# Autodesk Inventor assembly: ArmWithBase
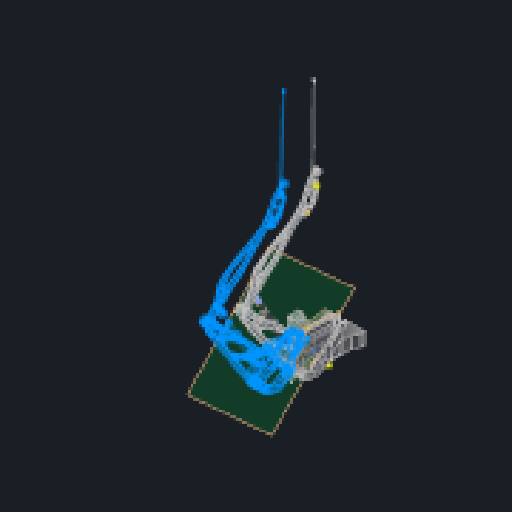
[picture p0: Inventor's stored thumbnail of the model, 512x512]
Saved by Autodesk Inventor 2025.2 (Build 292293000, 293)
## iProperties
Created: 2025-01-19
Part Number: ArmWithBase
Document SubType Name: Assembly
Designer: valer
Author: valer
## Documents named in this file (4)
- C:\Users\valer\Desktop\str1ker\cad\ArmFrontRight.iam
- C:\Users\valer\Desktop\str1ker\cad\ArmBase.iam
- C:\Users\valer\Desktop\str1ker\cad\Arm.iam
- C:\Users\valer\Desktop\str1ker\cad\ArmScapula.ipt
## Components (4 placed, 3 different names)
1. Base:1 [sub-assembly] — Mate:5, Mate:6, Mate:7, Mate:9, Mate:13, Mate:14, Mate:15
2. Arm:1 [sub-assembly] — Mate:5, Mate:6, Mate:8
3. ArmScapula:1 — Mate:9
4. ArmScapula:2 — Mate:13, Mate:14, Mate:15
## Relationships (8: Mate 8)
- Mate:5: Base:1 ↔ Arm:1
- Mate:6: Base:1 ↔ Arm:1
- Mate:7: Base:1
- Mate:8: Arm:1
- Mate:9: Base:1 ↔ ArmScapula:1
- Mate:13: Base:1 ↔ ArmScapula:2
- Mate:14: Base:1 ↔ ArmScapula:2
- Mate:15: Base:1 ↔ ArmScapula:2
